# Autodesk Inventor assembly: TR2 Arm
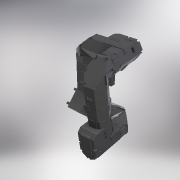
[picture p0: Inventor's stored thumbnail of the model, 180x180]
Saved by Autodesk Inventor 2017 (Build 210142000, 142)
## iProperties
Created: 2018-10-11
Part Number: TR2 Arm
Document SubType Name: Assembly
Designer: Zach
Author: Zach
## Documents named in this file (7)
- C:\Users\Dell\Documents\GitHub\tr2\Arm\Arm.iam
- C:\Users\Dell\Documents\GitHub\tr2\Gripper\Gripper.iam
- C:\Users\Dell\Documents\GitHub\tr2\Arm\TARM09b.ipt
- C:\Users\Dell\Documents\GitHub\tr2\Arm\TARM01b.ipt
- C:\Users\Dell\Documents\GitHub\tr2\Arm\TARM02b.ipt
- C:\Users\Dell\Documents\GitHub\tr2\Arm\TARM14.ipt
- C:\Users\Dell\Documents\GitHub\tr2\Actuator 1.2\Actuator 1.2.iam
## Components (12 placed, 6 different names)
1. TARM01b:1 — Mate:241, Mate:242, Mate:243, Mate:244, Mate:245, Mate:246
2. Gripper:1 [sub-assembly] — Mate:239, Mate:240
3. TARM09b:1 — Mate:186, Mate:187, Mate:188, Mate:221, Mate:222, Mate:223
4. TARM09b:2 — Mate:229, Mate:230, Mate:231, Mate:232, Mate:233
5. TARM02b:1 — Mate:186, Mate:187, Mate:188, Mate:247, Mate:248
6. TARM14:1 — Mate:224, Mate:225, Mate:226, Mate:227, Mate:228
7. TARM14:2 — Mate:234, Mate:235, Mate:236, Mate:237, Mate:238
8. Actuator 1.2:1 [sub-assembly] — Mate:221, Mate:222, Mate:223, Mate:224, Mate:225
9. Actuator 1.2:2 [sub-assembly] — Mate:226, Mate:227, Mate:228, Mate:229, Mate:230
10. Actuator 1.2:3 [sub-assembly] — Mate:231, Mate:232, Mate:233, Mate:234, Mate:235
11. Actuator 1.2:4 [sub-assembly] — Mate:236, Mate:237, Mate:238, Mate:239, Mate:240
12. Actuator 1.2:5 [sub-assembly] — Mate:244, Mate:245, Mate:246, Mate:247, Mate:248
## Relationships (31: Mate 31)
- Mate:186: TARM09b:1 ↔ TARM02b:1
- Mate:187: TARM09b:1 ↔ TARM02b:1
- Mate:188: TARM09b:1 ↔ TARM02b:1
- Mate:221: TARM09b:1 ↔ Actuator 1.2:1
- Mate:222: TARM09b:1 ↔ Actuator 1.2:1
- Mate:223: TARM09b:1 ↔ Actuator 1.2:1
- Mate:224: TARM14:1 ↔ Actuator 1.2:1
- Mate:225: TARM14:1 ↔ Actuator 1.2:1
- Mate:226: TARM14:1 ↔ Actuator 1.2:2
- Mate:227: TARM14:1 ↔ Actuator 1.2:2
- Mate:228: TARM14:1 ↔ Actuator 1.2:2
- Mate:229: TARM09b:2 ↔ Actuator 1.2:2
- Mate:230: TARM09b:2 ↔ Actuator 1.2:2
- Mate:231: TARM09b:2 ↔ Actuator 1.2:3
- Mate:232: TARM09b:2 ↔ Actuator 1.2:3
- Mate:233: TARM09b:2 ↔ Actuator 1.2:3
- Mate:234: TARM14:2 ↔ Actuator 1.2:3
- Mate:235: TARM14:2 ↔ Actuator 1.2:3
- Mate:236: TARM14:2 ↔ Actuator 1.2:4
- Mate:237: TARM14:2 ↔ Actuator 1.2:4
- Mate:238: TARM14:2 ↔ Actuator 1.2:4
- Mate:239: Gripper:1 ↔ Actuator 1.2:4
- Mate:240: Gripper:1 ↔ Actuator 1.2:4
- Mate:241: TARM01b:1
- Mate:242: TARM01b:1
- Mate:243: TARM01b:1
- Mate:244: TARM01b:1 ↔ Actuator 1.2:5
- Mate:245: TARM01b:1 ↔ Actuator 1.2:5
- Mate:246: TARM01b:1 ↔ Actuator 1.2:5
- Mate:247: TARM02b:1 ↔ Actuator 1.2:5
- Mate:248: TARM02b:1 ↔ Actuator 1.2:5
